# Autodesk Inventor assembly: Backplane
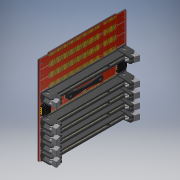
[picture p0: Inventor's stored thumbnail of the model, 180x180]
Saved by Autodesk Inventor 2018 (Build 220112000, 112)
## iProperties
Created: 2018-10-18
Part Number: Backplane
Document SubType Name: Assembly
Designer: Bradley
Author: Bradley
## Documents named in this file (8)
- C:\Users\Bradley\Documents\GitHub\CougSat1-Hardware\CougSat1-Backplane\CADModel\Native\Backplane.iam
- C:\Users\Bradley\Documents\GitHub\CougSat1-Hardware\CougSat1-Backplane\CADModel\Native\Backplane_PCB.ipt
- C:\Users\Bradley\Documents\GitHub\Resources\ComponentModels\Connectors\PicoLock-J-4.ipt
- C:\Users\Bradley\Documents\GitHub\Resources\ComponentModels\Connectors\PicoLock-P-4.ipt
- C:\Users\Bradley\Documents\GitHub\Resources\ComponentModels\Connectors\SODIMM-DDR.ipt
- C:\Users\Bradley\Documents\GitHub\Resources\ComponentModels\Electronics\Capacitor_1608-0.8mm.ipt
- C:\Users\Bradley\Documents\GitHub\Resources\ComponentModels\Electronics\Resistor_1608-0.5mm.ipt
- C:\Users\Bradley\Documents\GitHub\CougSat1-Hardware\CougSat1-Backplane\CADModel\Native\Backplane_CenterNut.ipt
## Components (15 placed, 7 different names)
1. Backplane_PCB:1 — Mate:5, Mate:6, Mate:9, Mate:10, Mate:11, Mate:12, Insert:17, Insert:18, Insert:19, Insert:20, Insert:21, Insert:22, Insert:23, Insert:30, Insert:31, Insert:32, Insert:33, Insert:34
2. Backplane_CenterNut:1 — Insert:17, Insert:18
3. PicoLock-J-4:1 — Mate:5, Flush:3, Mate:7
4. PicoLock-J-4:2 — Mate:6, Mate:8, Flush:4
5. PicoLock-P-4:1
6. PicoLock-P-4:2
7. SODIMM-DDR:1 — Insert:19, Insert:34
8. SODIMM-DDR:2 — Insert:20, Insert:33
9. SODIMM-DDR:3 — Insert:21, Insert:32
10. SODIMM-DDR:4 — Insert:22, Insert:31
11. SODIMM-DDR:5 — Insert:23, Insert:30
12. Capacitor_1608-0.8mm:1 — Mate:11, Mate:13, Mate:14
13. Capacitor_1608-0.8mm:2 — Mate:12, Mate:17, Flush:5
14. Resistor_1608-0.5mm:1 — Mate:9, Mate:15, Mate:16
15. Resistor_1608-0.5mm:2 — Mate:10, Mate:18, Flush:6
## Relationships (36: Mate 18, Insert 12, Flush 6)
- [Flush]: PicoLock-J-4:1 ↔ PicoLock-P-4:1
- [Mate]: PicoLock-J-4:1 ↔ PicoLock-P-4:1
- [Mate] (0.025 mm): PicoLock-J-4:1 ↔ PicoLock-P-4:1
- [Flush]: PicoLock-J-4:2 ↔ PicoLock-P-4:2
- [Mate]: PicoLock-J-4:2 ↔ PicoLock-P-4:2
- [Mate] (0.025 mm): PicoLock-J-4:2 ↔ PicoLock-P-4:2
- Mate:5: Backplane_PCB:1 ↔ PicoLock-J-4:1
- Mate:6: Backplane_PCB:1 ↔ PicoLock-J-4:2
- Flush:3: PicoLock-J-4:1
- Mate:7 (-32 mm): PicoLock-J-4:1
- Mate:8: PicoLock-J-4:2
- Flush:4 (32 mm): PicoLock-J-4:2
- Mate:9: Backplane_PCB:1 ↔ Resistor_1608-0.5mm:1
- Mate:10: Backplane_PCB:1 ↔ Resistor_1608-0.5mm:2
- Mate:11: Backplane_PCB:1 ↔ Capacitor_1608-0.8mm:1
- Mate:12: Backplane_PCB:1 ↔ Capacitor_1608-0.8mm:2
- Mate:13: Capacitor_1608-0.8mm:1
- Mate:14 (-9.4 mm): Capacitor_1608-0.8mm:1
- Mate:15: Resistor_1608-0.5mm:1
- Mate:16 (-7.5 mm): Resistor_1608-0.5mm:1
- Mate:17 (1.8 mm): Capacitor_1608-0.8mm:2
- Flush:5 (2.8 mm): Capacitor_1608-0.8mm:2
- Mate:18 (1.8 mm): Resistor_1608-0.5mm:2
- Flush:6 (4.7 mm): Resistor_1608-0.5mm:2
- Insert:17: Backplane_PCB:1 ↔ Backplane_CenterNut:1
- Insert:18: Backplane_PCB:1 ↔ Backplane_CenterNut:1
- Insert:19: Backplane_PCB:1 ↔ SODIMM-DDR:1
- Insert:20: Backplane_PCB:1 ↔ SODIMM-DDR:2
- Insert:21: Backplane_PCB:1 ↔ SODIMM-DDR:3
- Insert:22: Backplane_PCB:1 ↔ SODIMM-DDR:4
- Insert:23: Backplane_PCB:1 ↔ SODIMM-DDR:5
- Insert:30: Backplane_PCB:1 ↔ SODIMM-DDR:5
- Insert:31: Backplane_PCB:1 ↔ SODIMM-DDR:4
- Insert:32: Backplane_PCB:1 ↔ SODIMM-DDR:3
- Insert:33: Backplane_PCB:1 ↔ SODIMM-DDR:2
- Insert:34: Backplane_PCB:1 ↔ SODIMM-DDR:1
## Named parameters: d3_d9 = 0 mm, d4_d10 = 0 mm, d5_d11 = 0.025 mm
